# Autodesk Inventor assembly: tire_form 3
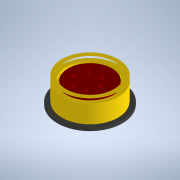
[picture p0: Inventor's stored thumbnail of the model, 180x180]
Saved by Autodesk Inventor 2022 (Build 260153000, 153)
## iProperties
Created: 2023-02-13
Part Number: tire_form 3
Document SubType Name: Assembly
Designer: akapu
Author: akapu
## Documents named in this file (4)
- C:\Users\akapu\OneDrive\Документы\maze bot\tire_form 3.iam
- C:\Users\akapu\OneDrive\Документы\maze bot\tire ring_3.ipt
- C:\Users\akapu\OneDrive\Документы\maze bot\tire_cap2.ipt
- C:\Users\akapu\OneDrive\Документы\maze bot\tire vtulka2.ipt
## Components (3 placed, 3 different names)
1. tire ring_3:1 — Совмещение:3, Совмещение:8
2. tire_cap2:1 — Совмещение:4, Совмещение:6, Совмещение:7
3. tire vtulka2:1 — Совмещение:3, Совмещение:4, Совмещение:5, Совмещение:6, Совмещение:7, Совмещение:8
## Relationships (6: Mate 6)
- Совмещение:3 [Mate]: tire ring_3:1 ↔ tire vtulka2:1
- Совмещение:4 [Mate]: tire_cap2:1 ↔ tire vtulka2:1
- Совмещение:5 [Mate]: tire vtulka2:1
- Совмещение:6 [Mate]: tire_cap2:1 ↔ tire vtulka2:1
- Совмещение:7 [Mate]: tire_cap2:1 ↔ tire vtulka2:1
- Совмещение:8 [Mate]: tire ring_3:1 ↔ tire vtulka2:1
